# Autodesk Inventor assembly: Hourglass
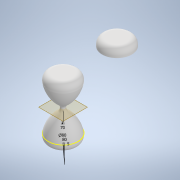
[picture p0: Inventor's stored thumbnail of the model, 180x180]
Saved by Autodesk Inventor 2020.2 (Build 242310000, 310)
## iProperties
Created: 2020-03-04
Part Number: Hourglass
Document SubType Name: Assembly
Designer: linus
Author: linus
## Documents named in this file (5)
- C:\Users\linus\Documents\Projects\Hourglass\Timglas\Hourglass.iam
- C:\Users\linus\Documents\Projects\Hourglass\Timglas\Timglas_main.ipt
- C:\Users\linus\Documents\Projects\Hourglass\Timglas\Top_and_Bottom.ipt
- C:\Users\linus\Documents\Projects\Hourglass\Timglas\Bottom.ipt
- C:\Users\linus\Documents\Projects\Hourglass\Timglas\Top.ipt
## Components (4 placed, 4 different names)
1. Timglas_main:1 — Insert:1, Insert:2
2. Top_and_Bottom:1
3. Top:1 — Insert:2
4. Bottom:1 — Insert:1
## Relationships (2: Insert 2)
- Insert:1: Timglas_main:1 ↔ Bottom:1
- Insert:2: Timglas_main:1 ↔ Top:1
